# Autodesk Inventor assembly: drop_center_wheel_MIR
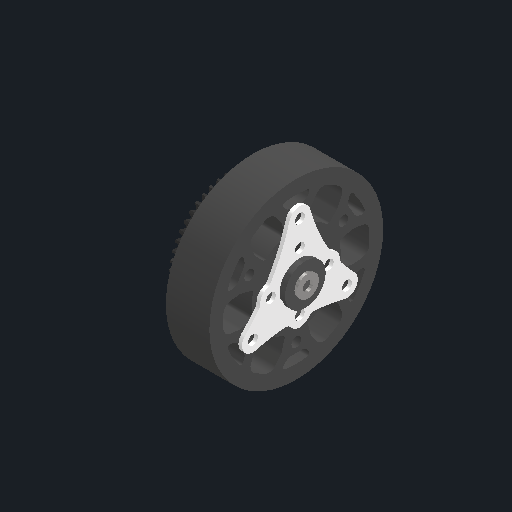
[picture p0: Inventor's stored thumbnail of the model, 512x512]
Saved by Autodesk Inventor 2024 (Build 280153000, 153)
## iProperties
Created: 2023-10-29
Part Number: drop_center_wheel_MIR
Document SubType Name: Assembly
Designer: avere
Author: avere
## Documents named in this file (12)
- C:\Users\avere\Documents\rbp_cad\zoomba_v0.1\chassis\mirrored_parts\drop_center_wheel_MIR.iam
- C:\Users\avere\Documents\rbp_cad\zoomba_v0.1\chassis\mirrored_parts\drop_center_hub_MIR.ipt
- C:\Users\avere\Documents\rbp_cad\VEX-CAD-Inventor-1.41\Motion\Wheels\Flex Wheels\3.000 Flex Wheel\3.000 60A .750.ipt
- C:\Users\avere\Documents\rbp_cad\VEX-CAD-Inventor-1.41\Motion\Wheels\Flex Wheels\3.000 Flex Wheel.ipt
- C:\Users\avere\Documents\rbp_cad\zoomba_v0.1\chassis\mirrored_parts\VersaHex Adapters .250_MIR.ipt
- C:\Users\avere\Documents\rbp_cad\VEX-CAD-Inventor-1.41\Motion\Spacers\Spacer Nylon .375 OD\NSpacer .375 OD x .250.ipt
- C:\Users\avere\Documents\rbp_cad\VEX-CAD-Inventor-1.41\Motion\Spacers\Spacer Nylon .375 OD.ipt
- C:\Users\avere\Documents\rbp_cad\zoomba_v0.1\chassis\mirrored_parts\washer_thin_MIR.ipt
- C:\Users\avere\Documents\rbp_cad\zoomba_v0.1\chassis\mirrored_parts\ls_48t_flat_MIR.ipt
- C:\Users\avere\Documents\rbp_cad\VEX-CAD-Inventor-1.41\Motion\Spacers\Washer Steel\SWasher .375 OD x .031250.ipt
- C:\Users\avere\Documents\rbp_cad\VEX-CAD-Inventor-1.41\Motion\Spacers\Washer Steel.ipt
- C:\Users\avere\Documents\rbp_cad\VEX-CAD-Inventor-1.41\Motion\Spacers\Washer Steel\SWasher .375 OD x .015625.ipt
## Components (10 placed, 8 different names)
1. drop_center_hub_MIR:1 — Insert:9, Mate:2
2. 3.000 60A .750:1 — Insert:9, Mate:2, Mate:3, Insert:3, Insert:4, Insert:8
3. drop_center_hub_MIR:2 — Mate:3, Insert:3
4. VersaHex Adapters .250_MIR:1 — Insert:4, Insert:13
5. NSpacer .375 OD x .250:1 — Insert:6, Insert:11
6. washer_thin_MIR:1 — Insert:6
7. VersaHex Adapters .250_MIR:2 — Insert:8, Insert:10
8. ls_48t_flat_MIR:1 — Insert:11, Insert:10
9. SWasher .375 OD x .031250:1 — Insert:13, Insert:12
10. SWasher .375 OD x .015625:2 — Insert:12
## Relationships (11: Insert 9, Mate 2)
- Insert:9: drop_center_hub_MIR:1 ↔ 3.000 60A .750:1
- Mate:2: drop_center_hub_MIR:1 ↔ 3.000 60A .750:1
- Mate:3: 3.000 60A .750:1 ↔ drop_center_hub_MIR:2
- Insert:3: 3.000 60A .750:1 ↔ drop_center_hub_MIR:2
- Insert:4 (1.5875 mm): 3.000 60A .750:1 ↔ VersaHex Adapters .250_MIR:1
- Insert:6: NSpacer .375 OD x .250:1 ↔ washer_thin_MIR:1
- Insert:8 (1.5875 mm): 3.000 60A .750:1 ↔ VersaHex Adapters .250_MIR:2
- Insert:11: NSpacer .375 OD x .250:1 ↔ ls_48t_flat_MIR:1
- Insert:10 (-3.175 mm): VersaHex Adapters .250_MIR:2 ↔ ls_48t_flat_MIR:1
- Insert:13: VersaHex Adapters .250_MIR:1 ↔ SWasher .375 OD x .031250:1
- Insert:12: SWasher .375 OD x .031250:1 ↔ SWasher .375 OD x .015625:2
